# Autodesk Inventor assembly: teststructure1
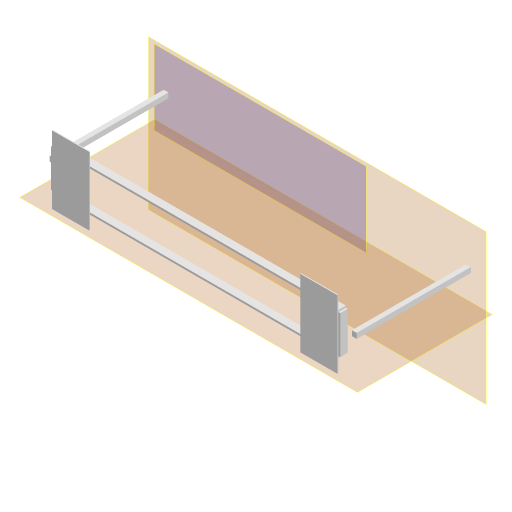
[picture p0: Inventor's stored thumbnail of the model, 512x512]
Saved by Autodesk Inventor 2024 (Build 280153000, 153)
## iProperties
Created: 2024-02-23
Part Number: teststructure1
Document SubType Name: Assembly
Designer: Frank
Author: Frank
## Documents named in this file (9)
- C:\Users\Cex\OneDrive\OneDrive - University of Bristol\Documents\Year_5\DP5\Agrivoltaicmodel\CAD\teststructure1.iam
- C:\Users\Cex\OneDrive\OneDrive - University of Bristol\Documents\Year_5\DP5\Agrivoltaicmodel\CAD\boxsectiontest.ipt
- C:\Users\Cex\OneDrive\OneDrive - University of Bristol\Documents\Year_5\DP5\Agrivoltaicmodel\CAD\testpanel.ipt
- C:\Users\Cex\OneDrive\OneDrive - University of Bristol\Documents\Year_5\DP5\Agrivoltaicmodel\CAD\boxsectiontestcross.ipt
- C:\Users\Cex\OneDrive\OneDrive - University of Bristol\Documents\Year_5\DP5\Agrivoltaicmodel\CAD\pylon.ipt
- C:\Users\Cex\OneDrive\OneDrive - University of Bristol\Documents\Year_5\DP5\Agrivoltaicmodel\CAD\boxsectiontest_MIR.ipt
- C:\Users\Cex\OneDrive\OneDrive - University of Bristol\Documents\Year_5\DP5\Agrivoltaicmodel\CAD\testpanel_MIR.ipt
- C:\Users\Cex\OneDrive\OneDrive - University of Bristol\Documents\Year_5\DP5\Agrivoltaicmodel\CAD\boxsectiontestcross_MIR.ipt
- C:\Users\Cex\OneDrive\OneDrive - University of Bristol\Documents\Year_5\DP5\Agrivoltaicmodel\CAD\pylon_MIR.ipt
## Components (15 placed, 8 different names)
1. boxsectiontest:1 — Mate:4, Flush:2, Mate:10, Flush:3, Mate:13, Mate:14, Mate:20
2. boxsectiontest:2 — Flush:1, Mate:9, Mate:11, Mate:12, Mate:15, Mate:18
3. testpanel:2 — Mate:18, Mate:20, Flush:5
4. boxsectiontestcross:1 — Mate:9, Mate:10, Flush:3, Mate:11, Mate:14, Mate:15, Mate:16, Mate:23
5. boxsectiontestcross:2 — Flush:1, Mate:4, Flush:2, Mate:8, Mate:12, Mate:13, Mate:22, Flush:6
6. pylon:1 — Mate:5, Mate:16, Flush:4, Mate:23
7. pylon:2 — Mate:6, Mate:8, Flush:4, Mate:21, Mate:22, Flush:6
8. boxsectiontest_MIR:1 — Mate:25, Mate:28, Flush:7, Mate:30, Mate:32, Flush:8, Mate:34, Flush:12, Mate:43, Mate:44
9. boxsectiontest_MIR:2 — Mate:26, Mate:27, Mate:29, Mate:31, Mate:33, Flush:9
10. testpanel_MIR:1 — Mate:24, Mate:25, Mate:26, Flush:12
11. boxsectiontestcross_MIR:1 — Mate:27, Mate:28, Mate:29, Flush:7, Mate:30, Mate:31, Mate:35, Mate:36
12. boxsectiontestcross_MIR:2 — Mate:32, Mate:33, Flush:8, Mate:34, Flush:9, Flush:10, Mate:38, Mate:40
13. pylon_MIR:1 — Mate:35, Mate:36, Mate:37, Flush:11
14. pylon_MIR:2 — Flush:10, Mate:38, Mate:39, Flush:11, Mate:40, Mate:41
15. testpanel_MIR:2 — Mate:42, Mate:43, Mate:44
## Relationships (50: Mate 38, Flush 12)
- Flush:1: boxsectiontest:2 ↔ boxsectiontestcross:2
- Mate:4 (2.5 mm): boxsectiontest:1 ↔ boxsectiontestcross:2
- Mate:5: pylon:1
- Mate:6: pylon:2
- Flush:2: boxsectiontest:1 ↔ boxsectiontestcross:2
- Mate:8: boxsectiontestcross:2 ↔ pylon:2
- Mate:9: boxsectiontest:2 ↔ boxsectiontestcross:1
- Mate:10: boxsectiontest:1 ↔ boxsectiontestcross:1
- Flush:3: boxsectiontest:1 ↔ boxsectiontestcross:1
- Mate:11 (2.5 mm): boxsectiontest:2 ↔ boxsectiontestcross:1
- Mate:12 (2.5 mm): boxsectiontest:2 ↔ boxsectiontestcross:2
- Mate:13 (2.5 mm): boxsectiontest:1 ↔ boxsectiontestcross:2
- Mate:14 (2.5 mm): boxsectiontest:1 ↔ boxsectiontestcross:1
- Mate:15 (2.5 mm): boxsectiontest:2 ↔ boxsectiontestcross:1
- Mate:16: boxsectiontestcross:1 ↔ pylon:1
- Flush:4: pylon:1 ↔ pylon:2
- Mate:18: boxsectiontest:2 ↔ testpanel:2
- Mate:20 (459.75 mm): boxsectiontest:1 ↔ testpanel:2
- Mate:21: pylon:2
- Flush:5: testpanel:2
- Mate:22 (146.8 mm): boxsectiontestcross:2 ↔ pylon:2
- Mate:23 (146.8 mm): boxsectiontestcross:1 ↔ pylon:1
- Flush:6 (574.75 mm): boxsectiontestcross:2 ↔ pylon:2
- Mate:24: testpanel_MIR:1
- Mate:25 (459.75 mm): boxsectiontest_MIR:1 ↔ testpanel_MIR:1
- Mate:26: boxsectiontest_MIR:2 ↔ testpanel_MIR:1
- Mate:27 (2.5 mm): boxsectiontest_MIR:2 ↔ boxsectiontestcross_MIR:1
- Mate:28 (2.5 mm): boxsectiontest_MIR:1 ↔ boxsectiontestcross_MIR:1
- Mate:29 (2.5 mm): boxsectiontest_MIR:2 ↔ boxsectiontestcross_MIR:1
- Flush:7: boxsectiontest_MIR:1 ↔ boxsectiontestcross_MIR:1
- Mate:30: boxsectiontest_MIR:1 ↔ boxsectiontestcross_MIR:1
- Mate:31: boxsectiontest_MIR:2 ↔ boxsectiontestcross_MIR:1
- Mate:32 (2.5 mm): boxsectiontest_MIR:1 ↔ boxsectiontestcross_MIR:2
- Mate:33 (2.5 mm): boxsectiontest_MIR:2 ↔ boxsectiontestcross_MIR:2
- Flush:8: boxsectiontest_MIR:1 ↔ boxsectiontestcross_MIR:2
- Mate:34 (2.5 mm): boxsectiontest_MIR:1 ↔ boxsectiontestcross_MIR:2
- Flush:9: boxsectiontest_MIR:2 ↔ boxsectiontestcross_MIR:2
- Mate:35 (146.8 mm): boxsectiontestcross_MIR:1 ↔ pylon_MIR:1
- Mate:36: boxsectiontestcross_MIR:1 ↔ pylon_MIR:1
- Mate:37: pylon_MIR:1
- Flush:10 (574.75 mm): boxsectiontestcross_MIR:2 ↔ pylon_MIR:2
- Mate:38 (146.8 mm): boxsectiontestcross_MIR:2 ↔ pylon_MIR:2
- Mate:39: pylon_MIR:2
- Flush:11: pylon_MIR:1 ↔ pylon_MIR:2
- Mate:40: boxsectiontestcross_MIR:2 ↔ pylon_MIR:2
- Mate:41: pylon_MIR:2
- Flush:12: boxsectiontest_MIR:1 ↔ testpanel_MIR:1
- Mate:42: testpanel_MIR:2
- Mate:43: boxsectiontest_MIR:1 ↔ testpanel_MIR:2
- Mate:44: boxsectiontest_MIR:1 ↔ testpanel_MIR:2
